# Autodesk Inventor assembly: ABD_LEFT_OP
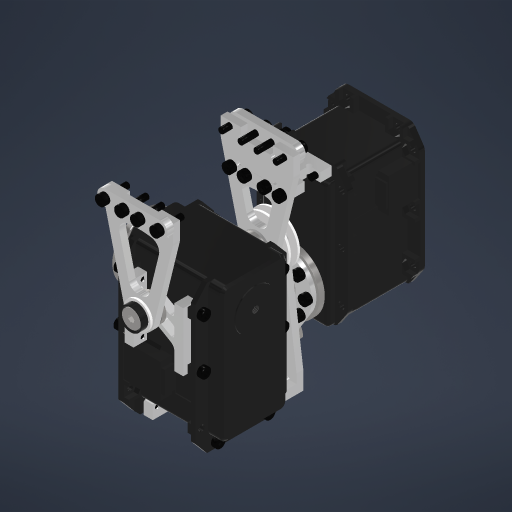
[picture p0: Inventor's stored thumbnail of the model, 512x512]
Saved by Autodesk Inventor 2024.3 (Build 283343000, 343)
## iProperties
Created: 2024-01-23
Part Number: ABD_LEFT_OP
Document SubType Name: Assembly
Designer: ASUS
Mass: 356.311 g
Surface Area: 603.891 cm^2
Volume: 181.117 cm^3
Author: ASUS
## Documents named in this file (21)
- C:\Users\ASUS\Desktop\test\v1_Frame\ABD_LEFT_OP.iam
- C:\Users\ASUS\Desktop\test\v1_Frame\Slider_crank_horn.ipt
- C:\Users\ASUS\Desktop\test\v1_Frame\Leg_joint_slider_frame.ipt
- C:\Users\ASUS\Desktop\test\v1_Frame\Roll_Fixation_L.ipt
- C:\Users\ASUS\Desktop\test\v1_Frame\Roll_Fixation_R.ipt
- C:\Users\ASUS\Desktop\test\v1_Frame\Roll_Fixation_Frame.ipt
- C:\Users\ASUS\Desktop\test\v1_Frame\Roll_Fixation_Frame_Back.ipt
- C:\Users\ASUS\Desktop\test\v1_Frame\Roll_Fixation_Frameto64.ipt
- C:\Users\ASUS\Desktop\test\v1_Frame\106_Slider_Fixation_MIR.ipt
- C:\Users\ASUS\Desktop\test\v1_Frame\hip joint fix washer.ipt
- C:\Users\ASUS\Desktop\test\Screw_Set\hip_joint_fix_washer_10mm_Set.iam
- C:\Users\ASUS\Desktop\test\Screw_Set\Roll_Fixation_Frame_8mm_Set.iam
- C:\Users\ASUS\Desktop\test\v1_Frame\MISUMI\CSH-ST-M2_5-8.ipt
- C:\Users\ASUS\Desktop\test\v1_Frame\Front_Frame_Fixer.iam
- C:\Users\ASUS\Desktop\test\v1_Frame\Crank_Slider_Fixer.iam
- C:\Users\ASUS\Desktop\test\v1_Frame\Rear_Frame_Fixer.iam
- C:\Users\ASUS\Desktop\test\Screw_Set\ABD_4mm_set.iam
- C:\Users\ASUS\Desktop\test\ROBOTIS(Inventor 2024 ver.)\DXL\MX-106T+idle.ipt.iam
- C:\Users\ASUS\Desktop\test\ROBOTIS(Inventor 2024 ver.)\DXL\MX-64T.ipt
- C:\Users\ASUS\Desktop\test\ROBOTIS(Inventor 2024 ver.)\HORN\64-106Horn.ipt
- MX-106T+idle.ipt
## Components (30 placed, 19 different names)
1. Slider_crank_horn:6 — 삽입:87, 메이트:327, 삽입:95, 삽입:99, 메이트:350
2. Roll_Fixation_Frame:8 — 메이트:210, 삽입:49, 삽입:50, 메이트:282, 삽입:90
3. Roll_Fixation_Frame_Back:6 — 메이트:210, 메이트:273, 메이트:274, 삽입:51, 메이트:279, 메이트:280, 메이트:281, 삽입:83, 삽입:86, 메이트:331, 메이트:332, 메이트:334, 삽입:100
4. Roll_Fixation_Frameto64:1 — 메이트:273, 메이트:274, 삽입:84, 삽입:85, 메이트:332, 삽입:98, 메이트:349
5. Roll_Fixation_L:6 — 각도:2, 메이트:333, 메이트:336, 메이트:337, 메이트:338, 메이트:339, 메이트:347
6. Roll_Fixation_R:2 — 각도:1, 삽입:96, 메이트:346
7. hip joint fix washer:1 — 삽입:49, 삽입:50, 메이트:280, 메이트:281, 메이트:282, 삽입:81, 메이트:325, 각도:3
8. hip joint fix washer:2 — 삽입:51, 메이트:279, 삽입:82, 메이트:326
9. Roll_Fixation_Frame_8mm_Set:4 [sub-assembly] — 메이트:337, 메이트:338, 메이트:339, 플러쉬:1, 메이트:340, 플러쉬:2
10. Roll_Fixation_Frame_8mm_Set:5 [sub-assembly] — 메이트:344, 플러쉬:2, 메이트:345, 메이트:346
11. CSH-ST-M2_5-8:9 — 삽입:78
12. CSH-ST-M2_5-8:10 — 삽입:79
13. Leg_joint_slider_frame:13 — 삽입:77, 메이트:322, 삽입:78, 삽입:79, 메이트:331, 메이트:352
14. 106_Slider_Fixation_MIR:2 — 삽입:77, 메이트:322, 메이트:343, 메이트:351
15. Roll_Fixation_Frame_8mm_Set:6 [sub-assembly] — 플러쉬:1, 메이트:341, 메이트:342, 메이트:351
16. hip_joint_fix_washer_10mm_Set:3 [sub-assembly] — 삽입:81, 메이트:325
17. hip_joint_fix_washer_10mm_Set:4 [sub-assembly] — 삽입:82, 메이트:326
18. CSH-ST-M2_5-8:11 — 삽입:86
19. CSH-ST-M2_5-8:12 — 삽입:83
20. CSH-ST-M2_5-8:13 — 삽입:85
21. CSH-ST-M2_5-8:14 — 삽입:84
22. ABD_4mm_set:2 [sub-assembly] — 삽입:87, 메이트:327
23. Front_Frame_Fixer:2 [sub-assembly] — 삽입:90, 각도:2, 메이트:333, 메이트:347
24. Rear_Frame_Fixer:2 [sub-assembly] — 각도:1, 메이트:334, 삽입:100
25. Crank_Slider_Fixer:1 [sub-assembly] — 삽입:95, 메이트:352
26. CSH-ST-M2_5-8:15 — 메이트:348, 메이트:349
27. CSH-ST-M2_5-8:16
28. MX-106T+idle.ipt:1 [sub-assembly] — 메이트:336, 삽입:96, 메이트:340, 메이트:341, 메이트:342, 메이트:343, 메이트:344, 메이트:345, 각도:4
29. MX-64T:1 — 삽입:97, 삽입:98, 메이트:348, 각도:4
30. 64-106Horn:1 — 삽입:97, 삽입:99, 메이트:350
## Relationships (58: Mate 32, Insert 20, Angle 4, Flush 2)
- 메이트:210 [Mate]: Roll_Fixation_Frame:8 ↔ Roll_Fixation_Frame_Back:6
- 메이트:273 [Mate]: Roll_Fixation_Frame_Back:6 ↔ Roll_Fixation_Frameto64:1
- 메이트:274 [Mate]: Roll_Fixation_Frame_Back:6 ↔ Roll_Fixation_Frameto64:1
- 삽입:49 [Insert]: Roll_Fixation_Frame:8 ↔ hip joint fix washer:1
- 삽입:50 [Insert]: Roll_Fixation_Frame:8 ↔ hip joint fix washer:1
- 삽입:51 [Insert]: Roll_Fixation_Frame_Back:6 ↔ hip joint fix washer:2
- 메이트:279 [Mate]: Roll_Fixation_Frame_Back:6 ↔ hip joint fix washer:2
- 메이트:280 [Mate]: Roll_Fixation_Frame_Back:6 ↔ hip joint fix washer:1
- 메이트:281 [Mate]: Roll_Fixation_Frame_Back:6 ↔ hip joint fix washer:1
- 메이트:282 [Mate]: Roll_Fixation_Frame:8 ↔ hip joint fix washer:1
- 삽입:77 [Insert]: Leg_joint_slider_frame:13 ↔ 106_Slider_Fixation_MIR:2
- 메이트:322 [Mate]: Leg_joint_slider_frame:13 ↔ 106_Slider_Fixation_MIR:2
- 삽입:78 [Insert]: CSH-ST-M2_5-8:9 ↔ Leg_joint_slider_frame:13
- 삽입:79 [Insert]: CSH-ST-M2_5-8:10 ↔ Leg_joint_slider_frame:13
- 삽입:81 [Insert]: hip joint fix washer:1 ↔ hip_joint_fix_washer_10mm_Set:3
- 메이트:325 [Mate]: hip joint fix washer:1 ↔ hip_joint_fix_washer_10mm_Set:3
- 삽입:82 [Insert]: hip joint fix washer:2 ↔ hip_joint_fix_washer_10mm_Set:4
- 메이트:326 [Mate]: hip joint fix washer:2 ↔ hip_joint_fix_washer_10mm_Set:4
- 삽입:83 [Insert]: Roll_Fixation_Frame_Back:6 ↔ CSH-ST-M2_5-8:12
- 삽입:84 [Insert]: Roll_Fixation_Frameto64:1 ↔ CSH-ST-M2_5-8:14
- 삽입:85 [Insert]: Roll_Fixation_Frameto64:1 ↔ CSH-ST-M2_5-8:13
- 삽입:86 [Insert]: Roll_Fixation_Frame_Back:6 ↔ CSH-ST-M2_5-8:11
- 삽입:87 [Insert]: Slider_crank_horn:6 ↔ ABD_4mm_set:2
- 메이트:327 [Mate]: Slider_crank_horn:6 ↔ ABD_4mm_set:2
- 삽입:90 [Insert]: Roll_Fixation_Frame:8 ↔ Front_Frame_Fixer:2
- 메이트:331 [Mate]: Roll_Fixation_Frame_Back:6 ↔ Leg_joint_slider_frame:13
- 메이트:332 [Mate]: Roll_Fixation_Frame_Back:6 ↔ Roll_Fixation_Frameto64:1
- 삽입:95 [Insert]: Slider_crank_horn:6 ↔ Crank_Slider_Fixer:1
- 각도:1 [Angle] (0 deg): Roll_Fixation_R:2 ↔ Rear_Frame_Fixer:2
- 각도:2 [Angle] (0 deg): Roll_Fixation_L:6 ↔ Front_Frame_Fixer:2
- 메이트:333 [Mate]: Roll_Fixation_L:6 ↔ Front_Frame_Fixer:2
- 메이트:334 [Mate]: Roll_Fixation_Frame_Back:6 ↔ Rear_Frame_Fixer:2
- 각도:3 [Angle] (0 deg): hip joint fix washer:1
- 메이트:336 [Mate] (0.5 mm): Roll_Fixation_L:6 ↔ MX-106T+idle.ipt:1
- 메이트:337 [Mate] (3.55 mm): Roll_Fixation_L:6 ↔ Roll_Fixation_Frame_8mm_Set:4
- 메이트:338 [Mate]: Roll_Fixation_L:6 ↔ Roll_Fixation_Frame_8mm_Set:4
- 메이트:339 [Mate]: Roll_Fixation_L:6 ↔ Roll_Fixation_Frame_8mm_Set:4
- 플러쉬:1 [Flush]: Roll_Fixation_Frame_8mm_Set:4 ↔ Roll_Fixation_Frame_8mm_Set:6
- 삽입:96 [Insert] (0.5 mm): Roll_Fixation_R:2 ↔ MX-106T+idle.ipt:1
- 메이트:340 [Mate]: Roll_Fixation_Frame_8mm_Set:4 ↔ MX-106T+idle.ipt:1
- 메이트:341 [Mate]: Roll_Fixation_Frame_8mm_Set:6 ↔ MX-106T+idle.ipt:1
- 메이트:342 [Mate]: Roll_Fixation_Frame_8mm_Set:6 ↔ MX-106T+idle.ipt:1
- 메이트:343 [Mate] (0.5 mm): 106_Slider_Fixation_MIR:2 ↔ MX-106T+idle.ipt:1
- 메이트:344 [Mate]: Roll_Fixation_Frame_8mm_Set:5 ↔ MX-106T+idle.ipt:1
- 플러쉬:2 [Flush]: Roll_Fixation_Frame_8mm_Set:4 ↔ Roll_Fixation_Frame_8mm_Set:5
- 메이트:345 [Mate]: Roll_Fixation_Frame_8mm_Set:5 ↔ MX-106T+idle.ipt:1
- 메이트:346 [Mate]: Roll_Fixation_R:2 ↔ Roll_Fixation_Frame_8mm_Set:5
- 메이트:347 [Mate]: Roll_Fixation_L:6 ↔ Front_Frame_Fixer:2
- 삽입:97 [Insert] (0.5 mm): MX-64T:1 ↔ 64-106Horn:1
- 삽입:98 [Insert]: Roll_Fixation_Frameto64:1 ↔ MX-64T:1
- 메이트:348 [Mate]: CSH-ST-M2_5-8:15 ↔ MX-64T:1
- 메이트:349 [Mate]: Roll_Fixation_Frameto64:1 ↔ CSH-ST-M2_5-8:15
- 삽입:99 [Insert]: Slider_crank_horn:6 ↔ 64-106Horn:1
- 메이트:350 [Mate]: Slider_crank_horn:6 ↔ 64-106Horn:1
- 메이트:351 [Mate]: 106_Slider_Fixation_MIR:2 ↔ Roll_Fixation_Frame_8mm_Set:6
- 메이트:352 [Mate]: Leg_joint_slider_frame:13 ↔ Crank_Slider_Fixer:1
- 삽입:100 [Insert]: Roll_Fixation_Frame_Back:6 ↔ Rear_Frame_Fixer:2
- 각도:4 [Angle] (0 deg): MX-106T+idle.ipt:1 ↔ MX-64T:1
